# Autodesk Inventor assembly: zwischenstab
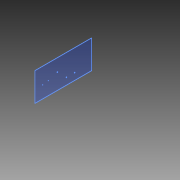
[picture p0: Inventor's stored thumbnail of the model, 180x180]
Saved by Autodesk Inventor 2013 (Build 170138000, 138)
## iProperties
Created: 2012-10-24
Part Number: zwischenstab
Document SubType Name: Assembly
Designer: fivef
Author: fivef
## Documents named in this file (3)
- D:\Dropbox\My Dropbox\Dokumente\Aktuell\Drinkmixer\zwischenstab.iam
- D:\Dropbox\My Dropbox\Dokumente\Aktuell\Drinkmixer\stab.ipt
- D:\Dropbox\My Dropbox\Dokumente\Aktuell\Drinkmixer\mutter.ipt
## Components (3 placed, 2 different names)
1. stab:1 — Fluchtend:1, Fluchtend:2, Passend:1, Passend:2
2. mutter:1 — Fluchtend:1
3. mutter:2 — Fluchtend:2, Passend:1, Passend:2
## Relationships (4: Flush 2, Mate 2)
- Fluchtend:1 [Flush]: stab:1 ↔ mutter:1
- Fluchtend:2 [Flush]: stab:1 ↔ mutter:2
- Passend:1 [Mate]: stab:1 ↔ mutter:2
- Passend:2 [Mate]: stab:1 ↔ mutter:2
